# Autodesk Inventor assembly: tandwiel_MIROR
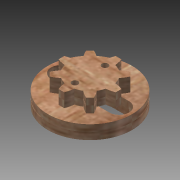
[picture p0: Inventor's stored thumbnail of the model, 180x180]
Saved by Autodesk Inventor 2015 (Build 190159000, 159)
## iProperties
Created: 2016-01-31
Part Number: tandwiel_MIROR
Document SubType Name: Assembly
Designer: david
Author: david
## Documents named in this file (3)
- Z:\gip\Inventor\generatie 7\Motor\tandwiel\tandwiel_MIROR.iam
- Z:\gip\Inventor\generatie 7\Motor\tandwiel\1_MIROR.ipt
- Z:\gip\Inventor\generatie 7\Motor\tandwiel\tandwiel(ja)_MIROR.ipt
## Components (4 placed, 2 different names)
1. 1_MIROR:1 — Flush:1, Mate:2, Mate:1
2. 1_MIROR:2 — Flush:1, Mate:2, Mate:1, Flush:2
3. tandwiel(ja)_MIROR:1 — Flush:2, Mate:4, Mate:3
4. tandwiel(ja)_MIROR:2 — Mate:4, Mate:3
## Relationships (6: Mate 5, Flush 1)
- Flush:1: 1_MIROR:1 ↔ 1_MIROR:2
- Mate:2: 1_MIROR:1 ↔ 1_MIROR:2
- Mate:1: 1_MIROR:1 ↔ 1_MIROR:2
- Flush:2 [Mate]: 1_MIROR:2 ↔ tandwiel(ja)_MIROR:1
- Mate:4: tandwiel(ja)_MIROR:1 ↔ tandwiel(ja)_MIROR:2
- Mate:3: tandwiel(ja)_MIROR:1 ↔ tandwiel(ja)_MIROR:2
